# Autodesk Inventor assembly: prototipo
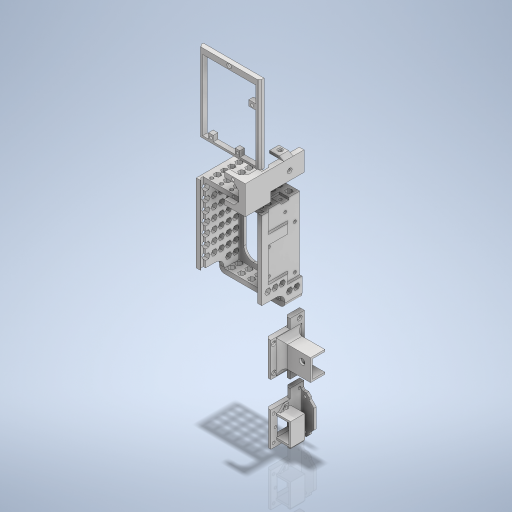
[picture p0: Inventor's stored thumbnail of the model, 512x512]
Saved by Autodesk Inventor 2024.3 (Build 283343000, 343)
## iProperties
Created: 2024-03-02
Part Number: prototipo
Document SubType Name: Assembly
Designer: joaov
Author: joaov
## Documents named in this file (7)
- D:\Downloads\IC\Bancada\prototipo_v2\prototipo_v2.iam
- D:\Downloads\IC\Bancada\prototipo_v2\corpo.ipt
- D:\Downloads\IC\Bancada\prototipo_v2\tampa.ipt
- D:\Downloads\IC\Bancada\prototipo_v2\bloco_aquecimento.ipt
- D:\Downloads\IC\Bancada\prototipo_v2\ventilador.ipt
- D:\Downloads\IC\Bancada\prototipo_v2\protetor_luz.ipt
- D:\Downloads\IC\Bancada\prototipo_v2\suporte_esquerdo.ipt
## Components (6 placed, 6 different names)
1. corpo:1 — Coincidente:2, Coincidente:3, Alinhado:3, Coincidente:4, Coincidente:5, Coincidente:6, Coincidente:9, Coincidente:10
2. tampa_1 — Coincidente:2, Coincidente:3
3. bloco_aquecimento:1 — Coincidente:9, Coincidente:10
4. ventilador:1 — Coincidente:5, Coincidente:6, Coincidente:7, Coincidente:8
5. protetor_luz:1 — Coincidente:7, Coincidente:8
6. suporte_esquerdo:1 — Alinhado:3, Coincidente:4
## Relationships (10: Mate 9, Flush 1)
- Coincidente:2 [Mate]: corpo:1 ↔ tampa_1
- Coincidente:3 [Mate]: corpo:1 ↔ tampa_1
- Alinhado:3 [Flush]: corpo:1 ↔ suporte_esquerdo:1
- Coincidente:4 [Mate]: corpo:1 ↔ suporte_esquerdo:1
- Coincidente:5 [Mate]: corpo:1 ↔ ventilador:1
- Coincidente:6 [Mate]: corpo:1 ↔ ventilador:1
- Coincidente:7 [Mate]: ventilador:1 ↔ protetor_luz:1
- Coincidente:8 [Mate]: ventilador:1 ↔ protetor_luz:1
- Coincidente:9 [Mate]: corpo:1 ↔ bloco_aquecimento:1
- Coincidente:10 [Mate]: corpo:1 ↔ bloco_aquecimento:1
